# Autodesk Inventor assembly: Assieme_coperchio
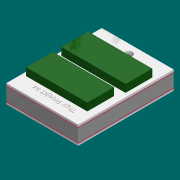
[picture p0: Inventor's stored thumbnail of the model, 180x180]
Saved by Autodesk Inventor 2020 (Build 240168000, 168)
## iProperties
Created: 2025-01-02
Part Number: Assieme_coperchio
Document SubType Name: Assembly
Designer: Nicola Milia
Author: Nicola Milia
## Documents named in this file (5)
- C:\Users\milit\Desktop\Progetti\Project THOR\Coperchio Sx V3\Assieme_coperchio.iam
- C:\Users\milit\Desktop\Progetti\Project THOR\Coperchio Sx V3\Struttura.ipt
- C:\Users\milit\Desktop\Progetti\Project THOR\Coperchio Sx V3\pcb.ipt
- C:\Users\milit\Desktop\Progetti\Project THOR\Coperchio Sx V3\tappo ingeriore.ipt
- C:\Users\milit\Desktop\Progetti\Project THOR\Coperchio Sx V3\tappo superiore.ipt
## Components (4 placed, 4 different names)
1. Struttura:1 — Allineato:2, Allineato:5, Allineato:6, Allineato:7
2. pcb:1 — Allineato:1, Allineato:2, Allineato:3, Allineato:4
3. tappo ingeriore:1 — Allineato:3, Allineato:4
4. tappo superiore:1 — Allineato:5, Allineato:6, Allineato:7
## Relationships (7: Flush 7)
- Allineato:1 [Flush]: pcb:1
- Allineato:2 [Flush]: Struttura:1 ↔ pcb:1
- Allineato:3 [Flush]: pcb:1 ↔ tappo ingeriore:1
- Allineato:4 [Flush]: pcb:1 ↔ tappo ingeriore:1
- Allineato:5 [Flush]: Struttura:1 ↔ tappo superiore:1
- Allineato:6 [Flush]: Struttura:1 ↔ tappo superiore:1
- Allineato:7 [Flush]: Struttura:1 ↔ tappo superiore:1
